# Autodesk Inventor assembly: cellSTORM_v2
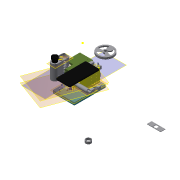
[picture p0: Inventor's stored thumbnail of the model, 180x180]
Saved by Autodesk Inventor 2019 (Build 230136000, 136)
## iProperties
Created: 2019-10-29
Part Number: cellSTORM_v2
Document SubType Name: Assembly
Designer: diederichbenedict
Author: diederichbenedict
## Documents named in this file (19)
- C:\Users\diederichbenedict\Dropbox\Dokumente\Promotion\PROJECTS\STORMoChip\INVENTOR\Nanoscopy-on-a-cheap\CHINESE\Workspace\cellSTORM_v2_china.iam
- C:\Users\diederichbenedict\Dropbox\Dokumente\Promotion\PROJECTS\STORMoChip\INVENTOR\Nanoscopy-on-a-cheap\Assembly_Lasergroup_wPickup_v1.iam
- C:\Users\diederichbenedict\Dropbox\Dokumente\Promotion\PROJECTS\STORMoChip\INVENTOR\Nanoscopy-on-a-cheap\100_chroma_HQ675_55.ipt
- C:\Users\diederichbenedict\Dropbox\Dokumente\Promotion\PROJECTS\STORMoChip\INVENTOR\Nanoscopy-on-a-cheap\02_Nanoscopy_Chip.ipt
- C:\Users\diederichbenedict\Dropbox\Dokumente\Promotion\PROJECTS\STORMoChip\INVENTOR\Nanoscopy-on-a-cheap\00_LASER_640nm.ipt
- C:\Users\diederichbenedict\Dropbox\Dokumente\Promotion\PROJECTS\STORMoChip\INVENTOR\Nanoscopy-on-a-cheap\00_KES400.iam
- C:\Users\diederichbenedict\Dropbox\Dokumente\Promotion\PROJECTS\STORMoChip\INVENTOR\Nanoscopy-on-a-cheap\00_Huawei_P20.ipt
- C:\Users\diederichbenedict\Dropbox\Dokumente\Promotion\PROJECTS\STORMoChip\INVENTOR\Nanoscopy-on-a-cheap\cellSTORM_Base_v0.ipt
- C:\Users\diederichbenedict\Dropbox\Dokumente\Promotion\PROJECTS\STORMoChip\INVENTOR\Nanoscopy-on-a-cheap\cellSTORM_Lasermount_v0.ipt
- C:\Users\diederichbenedict\Dropbox\Dokumente\Promotion\PROJECTS\STORMoChip\INVENTOR\Nanoscopy-on-a-cheap\cellSTORM_cellphone_objectivelens_mount.ipt
- C:\Users\diederichbenedict\Documents\Inventor\Content Center Files\R2019\en-US\DIN 912\DIN 912 - M3 x 0.5 x 25 x 18.ipt
- C:\Users\diederichbenedict\Dropbox\Dokumente\Promotion\PROJECTS\STORMoChip\INVENTOR\Nanoscopy-on-a-cheap\00_Ballmagnets_5mm.ipt
- C:\Users\diederichbenedict\Dropbox\Dokumente\Promotion\PROJECTS\STORMoChip\INVENTOR\Nanoscopy-on-a-cheap\00_Micrometer.ipt
- C:\Users\diederichbenedict\Dropbox\Dokumente\Promotion\PROJECTS\STORMoChip\INVENTOR\Nanoscopy-on-a-cheap\cellSTORM_Wheel_Micrometer.ipt
- C:\Users\diederichbenedict\Dropbox\Dokumente\Promotion\PROJECTS\STORMoChip\INVENTOR\Nanoscopy-on-a-cheap\cellSTORM_Spacerring_ocular.ipt
- C:\Users\diederichbenedict\Dropbox\Dokumente\Promotion\PROJECTS\STORMoChip\INVENTOR\Nanoscopy-on-a-cheap\cellSTORM_screw_ring_adjuster.ipt
- C:\Users\diederichbenedict\Dropbox\Dokumente\Promotion\PROJECTS\STORMoChip\INVENTOR\Nanoscopy-on-a-cheap\cellSTORM_coverslip_slide_adapter.ipt
- C:\Users\diederichbenedict\Dropbox\Dokumente\Promotion\PROJECTS\STORMoChip\INVENTOR\Nanoscopy-on-a-cheap\CHINESE\Workspace\00_XY_stage-Chinese_60x60-R1.iam
- C:\Users\diederichbenedict\Dropbox\Dokumente\Promotion\PROJECTS\STORMoChip\INVENTOR\Nanoscopy-on-a-cheap\Assembly_Eyepiece_Folded_longtube.iam
## Components (27 placed, 18 different names)
1. Assembly_Lasergroup_wPickup_v1:1 [sub-assembly]
2. 100_chroma_HQ675_55:1
3. DIN 912 - replaced by DIN EN ISO 4762 M3 x 25:2 — Mate:12
4. DIN 912 - replaced by DIN EN ISO 4762 M3 x 25:4 — Mate:11, Insert:20
5. DIN 912 - replaced by DIN EN ISO 4762 M3 x 25:5 — Mate:10, Insert:21
6. DIN 912 - replaced by DIN EN ISO 4762 M3 x 25:6 — Mate:9, Insert:19
7. 00_Ballmagnets_5mm:1 — Mate:12
8. 00_Ballmagnets_5mm:2 — Mate:9
9. 00_Ballmagnets_5mm:5 — Mate:11
10. 00_Ballmagnets_5mm:6 — Mate:10
11. 00_Ballmagnets_5mm:7
12. cellSTORM_Base_v0:1 — Insert:19, Insert:20, Insert:21, Angle:14, Angle:16, Flush:1, Insert:35, Angle:20
13. 00_LASER_640nm:1 — Mate:23, Angle:24, Insert:39
14. 02_Nanoscopy_Chip:1 — Angle:14
15. 00_Micrometer:1
16. cellSTORM_Wheel_Micrometer:1
17. 02_Nanoscopy_Chip:2 — Angle:16, Mate:25, Mate:26
18. cellSTORM_Spacerring_ocular:1
19. cellSTORM_screw_ring_adjuster:1 — Flush:1
20. cellSTORM_coverslip_slide_adapter:1
21. 00_XY_stage-Chinese_60x60-R1:2 [sub-assembly] — Insert:35, Angle:20, Insert:36, Angle:28
22. 00_KES400:1 [sub-assembly] — Mate:23, Angle:24, Mate:26
23. 00_Huawei_P20:1
24. Assembly_Eyepiece_Folded_longtube:1 [sub-assembly] — Mate:24, Mate:25
25. cellSTORM_Lasermount_v0:1 — Insert:36, Insert:37, Angle:25, Angle:26, Angle:27, Angle:28, Insert:39
26. 00_XY_stage-Chinese_60x60-R1:3 [sub-assembly] — Insert:37, Insert:38, Angle:25, Angle:27
27. cellSTORM_cellphone_objectivelens_mount:1 — Insert:38, Mate:24, Angle:26
## Relationships (25: Mate 8, Insert 8, Angle 8, Flush 1)
- Mate:9: DIN 912 - replaced by DIN EN ISO 4762 M3 x 25:6 ↔ 00_Ballmagnets_5mm:2
- Mate:10 (2 mm): DIN 912 - replaced by DIN EN ISO 4762 M3 x 25:5 ↔ 00_Ballmagnets_5mm:6
- Mate:11 (2 mm): DIN 912 - replaced by DIN EN ISO 4762 M3 x 25:4 ↔ 00_Ballmagnets_5mm:5
- Mate:12: DIN 912 - replaced by DIN EN ISO 4762 M3 x 25:2 ↔ 00_Ballmagnets_5mm:1
- Insert:19 (-10 mm): DIN 912 - replaced by DIN EN ISO 4762 M3 x 25:6 ↔ cellSTORM_Base_v0:1
- Insert:20 (10 mm): DIN 912 - replaced by DIN EN ISO 4762 M3 x 25:4 ↔ cellSTORM_Base_v0:1
- Insert:21 (10 mm): DIN 912 - replaced by DIN EN ISO 4762 M3 x 25:5 ↔ cellSTORM_Base_v0:1
- Angle:14 (0 deg): cellSTORM_Base_v0:1 ↔ 02_Nanoscopy_Chip:1
- Angle:16 (0 deg): cellSTORM_Base_v0:1 ↔ 02_Nanoscopy_Chip:2
- Flush:1: cellSTORM_Base_v0:1 ↔ cellSTORM_screw_ring_adjuster:1
- Insert:35: cellSTORM_Base_v0:1 ↔ 00_XY_stage-Chinese_60x60-R1:2
- Angle:20 (180 deg): cellSTORM_Base_v0:1 ↔ 00_XY_stage-Chinese_60x60-R1:2
- Mate:23: 00_LASER_640nm:1 ↔ 00_KES400:1
- Angle:24 (180 deg): 00_LASER_640nm:1 ↔ 00_KES400:1
- Insert:36: 00_XY_stage-Chinese_60x60-R1:2 ↔ cellSTORM_Lasermount_v0:1
- Insert:37: cellSTORM_Lasermount_v0:1 ↔ 00_XY_stage-Chinese_60x60-R1:3
- Insert:38: 00_XY_stage-Chinese_60x60-R1:3 ↔ cellSTORM_cellphone_objectivelens_mount:1
- Mate:24: Assembly_Eyepiece_Folded_longtube:1 ↔ cellSTORM_cellphone_objectivelens_mount:1
- Angle:25 (0 deg): cellSTORM_Lasermount_v0:1 ↔ 00_XY_stage-Chinese_60x60-R1:3
- Angle:26 (0 deg): cellSTORM_Lasermount_v0:1 ↔ cellSTORM_cellphone_objectivelens_mount:1
- Angle:27 (0 deg): cellSTORM_Lasermount_v0:1 ↔ 00_XY_stage-Chinese_60x60-R1:3
- Angle:28 (0 deg): 00_XY_stage-Chinese_60x60-R1:2 ↔ cellSTORM_Lasermount_v0:1
- Mate:25: 02_Nanoscopy_Chip:2 ↔ Assembly_Eyepiece_Folded_longtube:1
- Mate:26: 02_Nanoscopy_Chip:2 ↔ 00_KES400:1
- Insert:39: 00_LASER_640nm:1 ↔ cellSTORM_Lasermount_v0:1
